# Autodesk Inventor assembly: Cylinder, Bi-directional
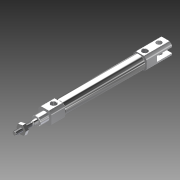
[picture p0: Inventor's stored thumbnail of the model, 180x180]
Saved by Autodesk Inventor 2014 SP1 (Build 180222100, 222)
## iProperties
Created: 2011-03-21
Part Number: Cylinder, Bi-directional
Document SubType Name: Assembly
Designer: Jordan
Translation Standard: STEP AP203
FileName: Cylinder, Bi-directional.iam
PreProcessor: SolidWorks 2007
PostProcessor: Build: 239, Release: 2011 RTM - Date: Wed 02/17/2010
Sent Units: millimeter
Uncertainty: 1e-05
Author: Jordan
## Documents named in this file (5)
- C:\Users\Ryan\Desktop\sw\lib\Aperture VEX CAD Library\Pnuematics\Cylinder, Bi-directional.iam
- C:\Users\Ryan\Desktop\sw\lib\Aperture VEX CAD Library\Pnuematics\Cylinder, Bi-directional-Parts\Nut 8-32 Hex.ipt
- C:\Users\Ryan\Desktop\sw\lib\Aperture VEX CAD Library\Pnuematics\Cylinder, Bi-directional-Parts\Rod.ipt
- C:\Users\Ryan\Desktop\sw\lib\Aperture VEX CAD Library\Pnuematics\Cylinder, Bi-directional-Parts\Body.ipt
- C:\Users\Ryan\Desktop\sw\lib\Aperture VEX CAD Library\Pnuematics\Cylinder, Bi-directional-Parts\Pin.ipt
## Components (4 placed, 4 different names)
1. Nut 8-32 Hex:1 — Flush:2, Mate:4
2. Rod:1 — Mate:3, Flush:1, Flush:2, Mate:4
3. Body:1 — Mate:1, Mate:2, Mate:3, Flush:1
4. Pin:1 — Mate:1, Mate:2
## Relationships (6: Mate 4, Flush 2)
- Mate:1: Body:1 ↔ Pin:1
- Mate:2: Body:1 ↔ Pin:1
- Mate:3: Rod:1 ↔ Body:1
- Flush:1 (-20 mm): Rod:1 ↔ Body:1
- Flush:2 (6.103 mm): Nut 8-32 Hex:1 ↔ Rod:1
- Mate:4: Nut 8-32 Hex:1 ↔ Rod:1
